# Autodesk Inventor assembly: Formule_sestava
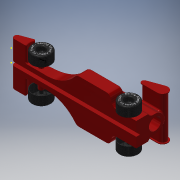
[picture p0: Inventor's stored thumbnail of the model, 180x180]
Saved by Autodesk Inventor 2018 (Build 220112000, 112)
## iProperties
Created: 2023-12-05
Part Number: Formule_sestava
Material: Všeobecné
Document SubType Name: Assembly
Designer: 42073
Author: 42073
## Documents named in this file (5)
- C:\Users\42073\Documents\2_Škola\inventor\Formule_sestava.iam
- C:\Users\42073\Documents\2_Škola\inventor\Telo_zavodnicky.ipt
- C:\Users\42073\Documents\2_Škola\inventor\naprava.ipt
- C:\Users\42073\Documents\2_Škola\inventor\kolo.ipt
- C:\Users\42073\Documents\2_Škola\inventor\pojistny_krouzek.ipt
## Components (9 placed, 4 different names)
1. Telo_zavodnicky:1 — Proti sobě:1, Proti sobě:2, Proti sobě:3, Proti sobě:4, Proti sobě:5, Proti sobě:6, Proti sobě:8
2. naprava:1 — Proti sobě:9, Proti sobě:11, Proti sobě:14
3. naprava:2 — Proti sobě:10, Proti sobě:12, Proti sobě:13
4. kolo:1 — Proti sobě:1, Proti sobě:6, Proti sobě:10, Proti sobě:12
5. kolo:2 — Proti sobě:2, Proti sobě:7, Proti sobě:8, Proti sobě:9, Proti sobě:11
6. kolo:3 — Proti sobě:4, Proti sobě:5
7. kolo:4 — Proti sobě:3, Proti sobě:7
8. pojistny_krouzek:1 — Proti sobě:13
9. pojistny_krouzek:2 — Proti sobě:14
## Relationships (14: Mate 14)
- Proti sobě:1 [Mate]: Telo_zavodnicky:1 ↔ kolo:1
- Proti sobě:2 [Mate]: Telo_zavodnicky:1 ↔ kolo:2
- Proti sobě:3 [Mate]: Telo_zavodnicky:1 ↔ kolo:4
- Proti sobě:4 [Mate]: Telo_zavodnicky:1 ↔ kolo:3
- Proti sobě:5 [Mate]: Telo_zavodnicky:1 ↔ kolo:3
- Proti sobě:6 [Mate]: Telo_zavodnicky:1 ↔ kolo:1
- Proti sobě:7 [Mate]: kolo:2 ↔ kolo:4
- Proti sobě:8 [Mate]: Telo_zavodnicky:1 ↔ kolo:2
- Proti sobě:9 [Mate]: naprava:1 ↔ kolo:2
- Proti sobě:10 [Mate]: naprava:2 ↔ kolo:1
- Proti sobě:11 [Mate]: naprava:1 ↔ kolo:2
- Proti sobě:12 [Mate]: naprava:2 ↔ kolo:1
- Proti sobě:13 [Mate]: naprava:2 ↔ pojistny_krouzek:1
- Proti sobě:14 [Mate]: naprava:1 ↔ pojistny_krouzek:2
